# Autodesk Inventor assembly: NixieClock
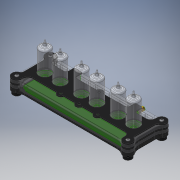
[picture p0: Inventor's stored thumbnail of the model, 180x180]
Saved by Autodesk Inventor 2017 (Build 210142000, 142)
## iProperties
Created: 2017-04-18
Part Number: NixieClock
Document SubType Name: Assembly
Designer: jeffkub
Author: jeffkub
## Documents named in this file (12)
- C:\Projects\nixie-clock\mechanical\NixieClock.iam
- C:\Projects\nixie-clock\mechanical\Base1.ipt
- C:\Projects\nixie-clock\mechanical\Base2.ipt
- C:\Projects\nixie-clock\mechanical\PCB.iam
- C:\Projects\nixie-clock\mechanical\Side.iam
- C:\Projects\nixie-clock\mechanical\Top.ipt
- C:\Projects\nixie-clock\mechanical\Cover.ipt
- C:\Projects\nixie-clock\mechanical\Front.ipt
- C:\Projects\nixie-clock\mechanical\Back.ipt
- C:\Projects\nixie-clock\mechanical\Bumper.ipt
- C:\Projects\nixie-clock\mechanical\M3x25mm.ipt
- C:\Projects\nixie-clock\mechanical\M3Nut.ipt
## Components (21 placed, 11 different names)
1. Base1:1 — Flush:1, Flush:2, Flush:3, Mate:1, Mate:16, Mate:17, Mate:18, Mate:19, Mate:20, Mate:21, Mate:22, Mate:23
2. Base2:1 — Mate:1, Flush:4, Flush:5, Mate:2, Mate:4, Mate:6, Mate:8, Mate:9, Mate:11, Mate:14
3. PCB:1 [sub-assembly] — Mate:2, Flush:6, Flush:7
4. Side:1 [sub-assembly] — Mate:4, Angle:1, Mate:7, Flush:11, Mate:8, Mate:13
5. Side:2 [sub-assembly] — Mate:6, Angle:2, Mate:9, Mate:15
6. Top:1 — Flush:8, Flush:9, Mate:7, Mate:10
7. Cover:1 — Flush:10, Flush:12, Flush:13, Mate:10, Mate:24, Mate:25, Mate:26, Mate:27, Mate:28, Mate:29, Mate:30, Mate:31
8. Front:1 — Mate:11, Mate:13, Flush:14
9. Back:1 — Flush:15, Mate:14, Mate:15
10. Bumper:1 — Mate:16, Mate:22, Mate:33
11. Bumper:2 — Mate:17, Mate:23, Mate:39
12. Bumper:3 — Mate:18, Mate:21, Mate:38
13. Bumper:4 — Mate:19, Mate:20, Mate:37
14. M3x25mm:1 — Mate:24, Mate:25, Mate:32
15. M3x25mm:2 — Mate:26, Mate:31, Mate:34
16. M3x25mm:3 — Mate:28, Mate:29, Mate:35
17. M3x25mm:4 — Mate:27, Mate:30, Mate:36
18. M3Nut:1 — Mate:32, Mate:33
19. M3Nut:2 — Mate:34, Mate:39
20. M3Nut:3 — Mate:36, Mate:37
21. M3Nut:4 — Mate:35, Mate:38
## Relationships (53: Mate 36, Flush 15, Angle 2)
- Flush:1: Base1:1
- Flush:2: Base1:1
- Flush:3: Base1:1
- Mate:1: Base1:1 ↔ Base2:1
- Flush:4: Base2:1
- Flush:5: Base2:1
- Mate:2: Base2:1 ↔ PCB:1
- Flush:6: PCB:1
- Flush:7: PCB:1
- Mate:4: Base2:1 ↔ Side:1
- Angle:1 (0 deg): Side:1
- Mate:6: Base2:1 ↔ Side:2
- Angle:2 (180 deg): Side:2
- Flush:8: Top:1
- Flush:9: Top:1
- Mate:7: Side:1 ↔ Top:1
- Flush:10: Cover:1
- Flush:11: Side:1
- Mate:8: Base2:1 ↔ Side:1
- Mate:9: Base2:1 ↔ Side:2
- Flush:12: Cover:1
- Flush:13: Cover:1
- Mate:10: Top:1 ↔ Cover:1
- Mate:11 (0.05 mm): Base2:1 ↔ Front:1
- Mate:13 (0.1 mm): Side:1 ↔ Front:1
- Flush:14: Front:1
- Flush:15: Back:1
- Mate:14 (0.05 mm): Base2:1 ↔ Back:1
- Mate:15 (0.1 mm): Side:2 ↔ Back:1
- Mate:16: Base1:1 ↔ Bumper:1
- Mate:17: Base1:1 ↔ Bumper:2
- Mate:18: Base1:1 ↔ Bumper:3
- Mate:19: Base1:1 ↔ Bumper:4
- Mate:20: Base1:1 ↔ Bumper:4
- Mate:21: Base1:1 ↔ Bumper:3
- Mate:22: Base1:1 ↔ Bumper:1
- Mate:23: Base1:1 ↔ Bumper:2
- Mate:24: Cover:1 ↔ M3x25mm:1
- Mate:25: Cover:1 ↔ M3x25mm:1
- Mate:26: Cover:1 ↔ M3x25mm:2
- Mate:27: Cover:1 ↔ M3x25mm:4
- Mate:28: Cover:1 ↔ M3x25mm:3
- Mate:29: Cover:1 ↔ M3x25mm:3
- Mate:30: Cover:1 ↔ M3x25mm:4
- Mate:31: Cover:1 ↔ M3x25mm:2
- Mate:32: M3x25mm:1 ↔ M3Nut:1
- Mate:33: Bumper:1 ↔ M3Nut:1
- Mate:34: M3x25mm:2 ↔ M3Nut:2
- Mate:35: M3x25mm:3 ↔ M3Nut:4
- Mate:36: M3x25mm:4 ↔ M3Nut:3
- Mate:37: Bumper:4 ↔ M3Nut:3
- Mate:38: Bumper:3 ↔ M3Nut:4
- Mate:39: Bumper:2 ↔ M3Nut:2
